# Autodesk Inventor assembly: Leg V4
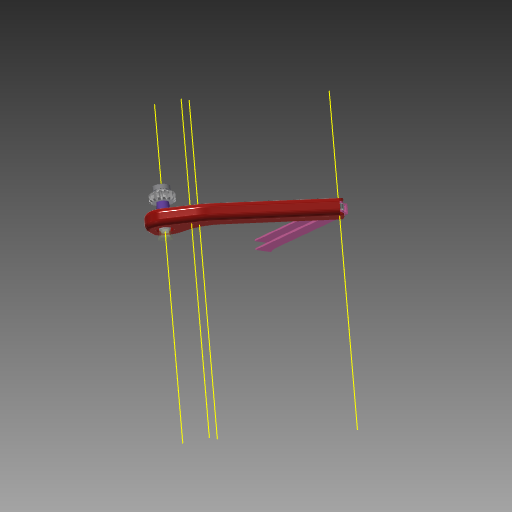
[picture p0: Inventor's stored thumbnail of the model, 512x512]
Saved by Autodesk Inventor 2019.1 (Build 231200000, 200)
## iProperties
Created: 2018-11-28
Part Number: Leg V4
Material: Generisch
Document SubType Name: Assembly
Designer: JochenAlt
Author: JochenAlt
## Documents named in this file (12)
- D:\Projects\Ondine\CAD\Leg\Leg V4.iam
- D:\Projects\Ondine\CAD\Leg\Leg V4.ipt
- D:\Projects\Ondine\CAD\Leg\Leg Inner V4.ipt
- D:\Projects\Ondine\CAD\Leg\LegInnerGear\Synchrone Riemenscheibe21.ipt
- D:\Projects\Ondine\CAD\Leg\LegInnerGear\Synchrone Riemenscheibe11.ipt
- D:\Projects\Ondine\CAD\Leg\LegInnerGear\Flache Riemenscheibe11.ipt
- D:\Projects\Ondine\CAD\Leg\LegInnerGear\Synchrone Riemenscheibe31.ipt
- D:\Projects\Ondine\CAD\Leg\Schnecke\Schneckenrad1.ipt
- D:\Projects\Ondine\CAD\Leg\LegInnerGear\gearNotch.ipt
- D:\Projects\Ondine\CAD\Bearings\W 61700 X-2RS1.iam
- D:\Projects\Ondine\CAD\Leg\LegInnerGear\Zahnriemen1.ipt
- D:\Projects\Ondine\CAD\Bearings\W 617_3.iam
## Components (12 placed, 10 different names)
1. Leg:1 — Passend:23, Winkel:3, Passend:40, Passend:60, Passend:64, Passend:65, Passend:68, Passend:69, Passend:70, Passend:71, Passend:76, Passend:77
2. Leg:2 — Passend:68, Winkel:4, Passend:69, Passend:71, Passend:72
3. Synchrone Riemenscheibe2:1 — Drehung:1, Passend:60, Passend:62
4. Synchrone Riemenscheibe1:1 — Passend:65, Passend:77
5. Flache Riemenscheibe1:1 — Passend:64, Passend:76
6. Synchrone Riemenscheibe3:1 — Winkel:2, Passend:21, Passend:23, Drehung:1, Passend:73, Passend:78, Passend:79, Passend:80, Passend:82
7. WormPinon:1 — Winkel:3, Passend:40, Passend:44, Passend:45, Passend:61, Passend:70, Passend:81
8. LegGearNotch:1 — Winkel:2, Passend:21, Winkel:4, Passend:80
9. W 61700 X-2RS1:2 [sub-assembly] — Passend:44, Passend:45
10. Zahnriemen:1 — Passend:61, Passend:62, Passend:72
11. W 61700 X-2RS1:3 [sub-assembly] — Passend:73, Passend:82
12. W 617_3:1 [sub-assembly] — Passend:78, Passend:79, Passend:81
## Relationships (27: Mate 23, Angle 3, RelateRotation 1)
- Winkel:2 [Angle] (180 deg): Synchrone Riemenscheibe3:1 ↔ LegGearNotch:1
- Passend:21 [Mate]: Synchrone Riemenscheibe3:1 ↔ LegGearNotch:1
- Passend:23 [Mate]: Leg:1 ↔ Synchrone Riemenscheibe3:1
- Winkel:3 [Angle] (180 deg): Leg:1 ↔ WormPinon:1
- Passend:40 [Mate]: Leg:1 ↔ WormPinon:1
- Passend:44 [Mate]: WormPinon:1 ↔ W 61700 X-2RS1:2
- Passend:45 [Mate]: WormPinon:1 ↔ W 61700 X-2RS1:2
- Drehung:1 [RelateRotation] (1 ul): Synchrone Riemenscheibe2:1 ↔ Synchrone Riemenscheibe3:1
- Passend:60 [Mate]: Leg:1 ↔ Synchrone Riemenscheibe2:1
- Passend:61 [Mate]: WormPinon:1 ↔ Zahnriemen:1
- Passend:62 [Mate]: Synchrone Riemenscheibe2:1 ↔ Zahnriemen:1
- Passend:64 [Mate]: Leg:1 ↔ Flache Riemenscheibe1:1
- Passend:65 [Mate]: Leg:1 ↔ Synchrone Riemenscheibe1:1
- Passend:68 [Mate]: Leg:1 ↔ Leg:2
- Winkel:4 [Angle] (0 deg): Leg:2 ↔ LegGearNotch:1
- Passend:69 [Mate] (1 mm): Leg:1 ↔ Leg:2
- Passend:70 [Mate]: Leg:1 ↔ WormPinon:1
- Passend:71 [Mate] (1 mm): Leg:1 ↔ Leg:2
- Passend:72 [Mate] (1 mm): Leg:2 ↔ Zahnriemen:1
- Passend:73 [Mate]: Synchrone Riemenscheibe3:1 ↔ W 61700 X-2RS1:3
- Passend:76 [Mate] (0.5 mm): Leg:1 ↔ Flache Riemenscheibe1:1
- Passend:77 [Mate] (0.5 mm): Leg:1 ↔ Synchrone Riemenscheibe1:1
- Passend:78 [Mate]: Synchrone Riemenscheibe3:1 ↔ W 617_3:1
- Passend:79 [Mate]: Synchrone Riemenscheibe3:1 ↔ W 617_3:1
- Passend:80 [Mate]: Synchrone Riemenscheibe3:1 ↔ LegGearNotch:1
- Passend:81 [Mate]: WormPinon:1 ↔ W 617_3:1
- Passend:82 [Mate]: Synchrone Riemenscheibe3:1 ↔ W 61700 X-2RS1:3
